# Autodesk Inventor assembly: sg90 long claw
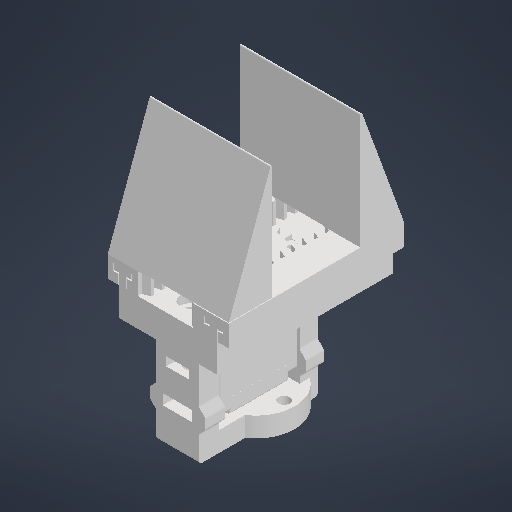
[picture p0: Inventor's stored thumbnail of the model, 512x512]
Saved by Autodesk Inventor 2026.1 (Build 301233020, 233B)
## iProperties
Created: 2025-06-09
Part Number: sg90 long claw
Document SubType Name: Assembly
Designer: gavin
Author: gavin
## Documents named in this file (6)
- F:\temp data disk\Github\6-DOF-Robot-Arm\3D-model\robot armT 2(CAD file)\sg90 long claw.iam
- F:\temp data disk\Github\6-DOF-Robot-Arm\3D-model\robot armT 2(CAD file)\9G Servo Motor SG90.ipt
- F:\temp data disk\Github\6-DOF-Robot-Arm\3D-model\robot armT 2(CAD file)\sg90 claw v2.ipt
- F:\temp data disk\Github\6-DOF-Robot-Arm\3D-model\robot armT 2(CAD file)\sg90 claw v2 gear m1.ipt
- F:\temp data disk\Github\6-DOF-Robot-Arm\3D-model\robot armT 2(CAD file)\sg90 claw v2 holder.ipt
- F:\temp data disk\Github\6-DOF-Robot-Arm\3D-model\robot armT 2(CAD file)\sg90 claw finger long.ipt
## Components (6 placed, 5 different names)
1. 9G Servo Motor SG90:1 — Mate:8, Mate:9, Mate:10
2. sg90 claw v2:1 — Mate:10, Flush:3, Flush:4
3. sg90 claw v2 gear m1:1
4. sg90 claw v2 holder:1 — Mate:8, Mate:9
5. sg90 claw finger long:1 — Flush:3
6. sg90 claw finger long:2 — Flush:4
## Relationships (14: Mate 10, Flush 4)
- [Flush]: 9G Servo Motor SG90:1 ↔ sg90 claw v2:1
- [Mate]: 9G Servo Motor SG90:1 ↔ sg90 claw v2 gear m1:1
- [Mate]: 9G Servo Motor SG90:1 ↔ sg90 claw v2 gear m1:1
- [Mate]: 9G Servo Motor SG90:1 ↔ sg90 claw v2:1
- [Flush]: 9G Servo Motor SG90:1 ↔ sg90 claw v2 holder:1
- [Mate]: sg90 claw v2:1 ↔ sg90 claw finger long:1
- [Mate] (0.2 mm): sg90 claw v2:1 ↔ sg90 claw finger long:1
- [Mate]: sg90 claw v2:1 ↔ sg90 claw finger long:2
- [Mate] (0.2 mm): sg90 claw v2:1 ↔ sg90 claw finger long:2
- Mate:8: 9G Servo Motor SG90:1 ↔ sg90 claw v2 holder:1
- Mate:9: 9G Servo Motor SG90:1 ↔ sg90 claw v2 holder:1
- Mate:10: 9G Servo Motor SG90:1 ↔ sg90 claw v2:1
- Flush:3: sg90 claw v2:1 ↔ sg90 claw finger long:1
- Flush:4: sg90 claw v2:1 ↔ sg90 claw finger long:2
